# Autodesk Inventor assembly: Assembly2
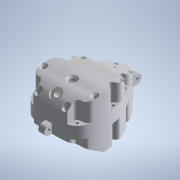
[picture p0: Inventor's stored thumbnail of the model, 180x180]
Saved by Autodesk Inventor 2021 (Build 250183000, 183)
## iProperties
Created: 2020-04-17
Part Number: Assembly2
Document SubType Name: Assembly
Designer: Matt
Author: Matt
## Documents named in this file (5)
- C:\Users\Derm\n95\v4\Assembly2.iam
- C:\Users\Derm\n95\v4\moldLid.ipt
- C:\Users\Derm\n95\v4\innerPositive.ipt
- C:\Users\Derm\n95\v4\lowerLeft.ipt
- C:\Users\Derm\n95\v4\lowerRight.ipt
## Components (4 placed, 4 different names)
1. moldLid:1 — Mate:3, Mate:5, Mate:6, Flush:1, Mate:8, Mate:9, Mate:11
2. innerPositive:1 — Mate:3, Flush:1, Mate:8, Mate:9
3. lowerLeft:1 — Mate:1, Mate:2, Mate:5, Mate:6, Mate:7, Mate:10
4. lowerRight:1 — Mate:1, Mate:2, Mate:7, Mate:10, Mate:11
## Relationships (11: Mate 10, Flush 1)
- Mate:1: lowerLeft:1 ↔ lowerRight:1
- Mate:2: lowerLeft:1 ↔ lowerRight:1
- Mate:3: moldLid:1 ↔ innerPositive:1
- Mate:5: moldLid:1 ↔ lowerLeft:1
- Mate:6: moldLid:1 ↔ lowerLeft:1
- Flush:1: moldLid:1 ↔ innerPositive:1
- Mate:7: lowerLeft:1 ↔ lowerRight:1
- Mate:8: moldLid:1 ↔ innerPositive:1
- Mate:9: moldLid:1 ↔ innerPositive:1
- Mate:10: lowerLeft:1 ↔ lowerRight:1
- Mate:11: moldLid:1 ↔ lowerRight:1
